# Autodesk Inventor assembly: 2.1mm DC Power Socket
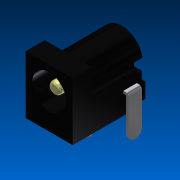
[picture p0: Inventor's stored thumbnail of the model, 180x180]
Saved by Autodesk Inventor 2013 (Build 170138000, 138)
## iProperties
Created: 2012-05-07
Document SubType Name: Assembly
Designer: sdarley
Project: 2.1mm DC Power Socket
Description: 2.1mm DC Power Socket
Author: sdarley
Title: 2.1mm DC Power Socket
Revision Number: 1
## Documents named in this file (6)
- C:\Users\sdarley\Documents\Inventor\General Design Work\2.1mm DC Power Socket\2.1mm DC Power Socket.iam
- C:\Users\sdarley\Documents\Inventor\General Design Work\2.1mm DC Power Socket\Components\2.1mm DC Power Socket Housing.ipt
- C:\Users\sdarley\Documents\Inventor\General Design Work\2.1mm DC Power Socket\Components\Terminal 3.ipt
- C:\Users\sdarley\Documents\Inventor\General Design Work\2.1mm DC Power Socket\Components\Terminal 1.ipt
- C:\Users\sdarley\Documents\Inventor\General Design Work\2.1mm DC Power Socket\Components\2.1mm DC Power Socket Pin.ipt
- C:\Users\sdarley\Documents\Inventor\General Design Work\2.1mm DC Power Socket\Components\Terminal 2.ipt
## Components (5 placed, 5 different names)
1. 2.1mm DC Power Socket Housing:1 — Mate:1, Mate:2, Flush:1, Mate:3, Flush:3, Flush:4, Flush:5, Mate:4, Mate:5, Flush:6, Mate:6, Mate:7, Flush:7
2. 2.1mm DC Power Socket Pin:1 — Flush:6, Mate:6, Mate:7
3. Terminal 1:1 — Flush:5, Mate:4, Mate:5, Mate:8, Flush:8
4. Terminal 2:1 — Flush:7, Mate:8, Flush:8
5. Terminal 3:1 — Mate:3, Flush:3, Flush:4
## Relationships (15: Mate 8, Flush 7)
- Mate:1: 2.1mm DC Power Socket Housing:1
- Mate:2: 2.1mm DC Power Socket Housing:1
- Flush:1: 2.1mm DC Power Socket Housing:1
- Mate:3: 2.1mm DC Power Socket Housing:1 ↔ Terminal 3:1
- Flush:3: 2.1mm DC Power Socket Housing:1 ↔ Terminal 3:1
- Flush:4 (2.25 mm): 2.1mm DC Power Socket Housing:1 ↔ Terminal 3:1
- Flush:5: 2.1mm DC Power Socket Housing:1 ↔ Terminal 1:1
- Mate:4: 2.1mm DC Power Socket Housing:1 ↔ Terminal 1:1
- Mate:5: 2.1mm DC Power Socket Housing:1 ↔ Terminal 1:1
- Flush:6: 2.1mm DC Power Socket Housing:1 ↔ 2.1mm DC Power Socket Pin:1
- Mate:6: 2.1mm DC Power Socket Housing:1 ↔ 2.1mm DC Power Socket Pin:1
- Mate:7: 2.1mm DC Power Socket Housing:1 ↔ 2.1mm DC Power Socket Pin:1
- Flush:7: 2.1mm DC Power Socket Housing:1 ↔ Terminal 2:1
- Mate:8 (-7.5 mm): Terminal 1:1 ↔ Terminal 2:1
- Flush:8: Terminal 1:1 ↔ Terminal 2:1
